# Autodesk Inventor assembly: sense3
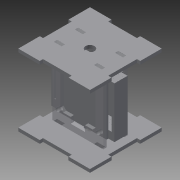
[picture p0: Inventor's stored thumbnail of the model, 180x180]
Saved by Autodesk Inventor 2013 (Build 170138000, 138)
## iProperties
Created: 2014-05-23
Part Number: sense3
Document SubType Name: Assembly
Designer: balogh
Author: balogh
## Documents named in this file (5)
- C:\Users\balogh\Documents\GitHub\sense_cube\sense3_inventor\sense3.iam
- C:\Users\balogh\Documents\GitHub\sense_cube\sense3_inventor\inside_box_top_bot.ipt
- C:\Users\balogh\Documents\GitHub\sense_cube\sense3_inventor\pcb_mount.ipt
- C:\Users\balogh\Documents\GitHub\sense_cube\sense3_inventor\battery_mount.ipt
- C:\Users\balogh\Documents\GitHub\sense_cube\sense3_inventor\pcb.ipt
## Components (10 placed, 4 different names)
1. inside_box_top_bot:1 — Angle:1, Mate:1, Mate:2, Mate:3, Mate:4, Flush:3, Flush:4
2. inside_box_top_bot:2 — Mate:5, Mate:6, Flush:1, Flush:2
3. pcb_mount:1 — Mate:3, Mate:4, Flush:2, Flush:4
4. pcb_mount:2 — Angle:1, Mate:1, Mate:2, Mate:5, Mate:6, Flush:1, Mate:12, Flush:3
5. battery_mount:1 — Insert:7, Insert:8, Insert:9, Insert:10
6. battery_mount:2 — Insert:9, Insert:10, Insert:11, Insert:12
7. battery_mount:3 — Insert:11, Insert:12, Insert:13, Insert:14
8. battery_mount:4 — Insert:13, Insert:14, Insert:15, Insert:16
9. pcb:1 — Insert:15, Insert:16
10. pcb:2 — Insert:7, Insert:8, Mate:12
## Relationships (22: Insert 10, Mate 7, Flush 4, Angle 1)
- Angle:1 (0 deg): inside_box_top_bot:1 ↔ pcb_mount:2
- Mate:1: inside_box_top_bot:1 ↔ pcb_mount:2
- Mate:2: inside_box_top_bot:1 ↔ pcb_mount:2
- Mate:3: inside_box_top_bot:1 ↔ pcb_mount:1
- Mate:4: inside_box_top_bot:1 ↔ pcb_mount:1
- Mate:5: inside_box_top_bot:2 ↔ pcb_mount:2
- Mate:6: inside_box_top_bot:2 ↔ pcb_mount:2
- Flush:1: inside_box_top_bot:2 ↔ pcb_mount:2
- Insert:7: battery_mount:1 ↔ pcb:2
- Insert:8: battery_mount:1 ↔ pcb:2
- Mate:12: pcb_mount:2 ↔ pcb:2
- Insert:9: battery_mount:1 ↔ battery_mount:2
- Insert:10: battery_mount:1 ↔ battery_mount:2
- Insert:11: battery_mount:2 ↔ battery_mount:3
- Insert:12: battery_mount:2 ↔ battery_mount:3
- Insert:13: battery_mount:3 ↔ battery_mount:4
- Insert:14: battery_mount:3 ↔ battery_mount:4
- Insert:15: battery_mount:4 ↔ pcb:1
- Insert:16: battery_mount:4 ↔ pcb:1
- Flush:2: inside_box_top_bot:2 ↔ pcb_mount:1
- Flush:3: inside_box_top_bot:1 ↔ pcb_mount:2
- Flush:4: inside_box_top_bot:1 ↔ pcb_mount:1
